# Autodesk Inventor assembly: XT-40
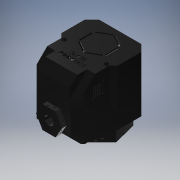
[picture p0: Inventor's stored thumbnail of the model, 180x180]
Saved by Autodesk Inventor 2017 SP1 (Build 210196100, 196)
## iProperties
Created: 2019-09-19
Part Number: XT-40
Document SubType Name: Assembly
Designer: Dell
Author: Dell
## Documents named in this file (17)
- C:\Users\Zach\Documents\GitHub\tr2\Actuator 2.0\XT-LG.iam
- C:\Users\Zach\Documents\GitHub\tr2\Actuator 2.0\AC01.ipt
- C:\Users\Zach\Documents\GitHub\tr2\Actuator 2.0\AC02.ipt
- C:\Users\Zach\Documents\GitHub\tr2\Actuator 2.0\AC05.ipt
- C:\Users\Zach\Documents\GitHub\tr2\Actuator 2.0\Slewing.iam
- C:\Users\Zach\Documents\GitHub\tr2\Actuator 2.0\Slip Ring.ipt
- C:\Users\Zach\Documents\GitHub\tr2\Actuator 2.0\8mm Mounting Hub.ipt
- C:\Users\Zach\Documents\GitHub\tr2\Actuator 2.0\AEAT-6012.ipt
- C:\Users\Zach\Documents\GitHub\tr2\Actuator 2.0\Series Elastic Gearbox 1.2\Series Elastic Gearbox 1.2.iam
- C:\Users\Zach\Documents\GitHub\tr2\Actuator 2.0\TS-40GZ7090.ipt
- C:\Users\Zach\Documents\GitHub\tr2\Actuator 2.0\Actuator 2.0\Design Accelerator\Spur Gears3.iam
- C:\Users\Zach\Documents\GitHub\tr2\Actuator 2.0\Actuator 2.0\Design Accelerator\Spur Gears4.iam
- C:\Users\Zach\Documents\GitHub\tr2\Actuator 2.0\Actuator 2.0\Design Accelerator\Spur Gears5.iam
- C:\Users\Zach\Documents\GitHub\tr2\Actuator 2.0\6201-2RS.ipt
- C:\Users\Zach\Documents\GitHub\tr2\Actuator 2.0\AC09.ipt
- C:\Users\Zach\Documents\GitHub\tr2\Actuator 2.0\AS 1110 - M6 x 35.ipt
- C:\Users\Zach\Documents\GitHub\tr2\Actuator 2.0\XT-LG-05.ipt
## Components (22 placed, 14 different names)
1. AC01:1 — Mate:3, Mate:4, Mate:5, Mate:9, Mate:139, Mate:140, Mate:141, Mate:142, Mate:145, Mate:146
2. AC02:1 — Mate:9, Mate:112, Mate:136, Mate:137, Mate:138, Mate:139, Mate:140, Mate:141, Mate:142, Mate:145, Mate:146, Mate:150, Mate:151, Mate:152, Mate:153, Mate:154, Mate:155, Mate:168, Mate:169, Mate:170, Mate:171, Mate:172, Mate:181, Mate:182, Mate:183, Mate:184, Flush:2, Flush:3
3. AC05:1 — Mate:6, Mate:7, Mate:8, Mate:23, Mate:24, Mate:25, Mate:90, Mate:91, Mate:92
4. Slewing:1 [sub-assembly] — Mate:3, Mate:4, Mate:5, Mate:6, Mate:7, Mate:8
5. Slip Ring:2 — Mate:23, Mate:24, Mate:25
6. 8mm Mounting Hub:1 — Mate:117, Mate:119
7. AEAT-6012:1 — Mate:151, Mate:158, Mate:162, Mate:163, Mate:164
8. AEAT-6012:2 — Mate:149, Mate:150, Mate:165, Mate:166, Mate:167
9. Series Elastic Gearbox 1.2:1 [sub-assembly] — Mate:90, Mate:91, Mate:92, Mate:113, Mate:114, Mate:116, Mate:120, Mate:134, Mate:143, Mate:156
10. TS-40GZ7090:1 — Mate:112, Mate:115, Mate:117, Mate:136, Mate:137, Mate:138, Mate:178, Mate:179, Mate:180
11. Spur Gears:1 [sub-assembly] — Mate:113, Mate:114, Mate:115, Mate:116, Mate:119, Mate:120, Rotation:1, Mate:144, Flush:1
12. Spur Gears:2 [sub-assembly] — Mate:134, Mate:143, Mate:144, Mate:156, Mate:158, Mate:174, Mate:177
13. Spur Gears:3 [sub-assembly] — Rotation:1, Mate:149, Flush:1, Mate:175, Mate:176
14. 6201-2RS:1 — Mate:154, Mate:155
15. 6201-2RS:2 — Mate:152, Mate:153
16. AC09:1 — Mate:162, Mate:163, Mate:164, Mate:165, Mate:166, Mate:167, Mate:168, Mate:169, Mate:170, Mate:171, Mate:172
17. AS 1110 - Metric M6 x 35:1 — Mate:174, Mate:177
18. AS 1110 - Metric M6 x 35:2 — Mate:175, Mate:176
19. AS 1110 - Metric M6 x 35:3 — Mate:178, Mate:181
20. AS 1110 - Metric M6 x 35:4 — Mate:179, Mate:182
21. AS 1110 - Metric M6 x 35:5 — Mate:180, Mate:183
22. XT-LG-05:1 — Mate:184, Flush:2, Flush:3
## Relationships (68: Mate 64, Flush 3, RelateRotation 1)
- Mate:3: AC01:1 ↔ Slewing:1
- Mate:4: AC01:1 ↔ Slewing:1
- Mate:5: AC01:1 ↔ Slewing:1
- Mate:6: AC05:1 ↔ Slewing:1
- Mate:7: AC05:1 ↔ Slewing:1
- Mate:8: AC05:1 ↔ Slewing:1
- Mate:9: AC01:1 ↔ AC02:1
- Mate:23: AC05:1 ↔ Slip Ring:2
- Mate:24 (5 mm): AC05:1 ↔ Slip Ring:2
- Mate:25: AC05:1 ↔ Slip Ring:2
- Mate:90: AC05:1 ↔ Series Elastic Gearbox 1.2:1
- Mate:91: AC05:1 ↔ Series Elastic Gearbox 1.2:1
- Mate:92: AC05:1 ↔ Series Elastic Gearbox 1.2:1
- Mate:112: AC02:1 ↔ TS-40GZ7090:1
- Mate:113: Series Elastic Gearbox 1.2:1 ↔ Spur Gears:1
- Mate:114: Series Elastic Gearbox 1.2:1 ↔ Spur Gears:1
- Mate:115: TS-40GZ7090:1 ↔ Spur Gears:1
- Mate:116: Series Elastic Gearbox 1.2:1 ↔ Spur Gears:1
- Mate:117: 8mm Mounting Hub:1 ↔ TS-40GZ7090:1
- Mate:119: 8mm Mounting Hub:1 ↔ Spur Gears:1
- Mate:120: Series Elastic Gearbox 1.2:1 ↔ Spur Gears:1
- Rotation:1 [RelateRotation] (1.0714 ul): Spur Gears:1 ↔ Spur Gears:3
- Mate:134: Series Elastic Gearbox 1.2:1 ↔ Spur Gears:2
- Mate:136: AC02:1 ↔ TS-40GZ7090:1
- Mate:137: AC02:1 ↔ TS-40GZ7090:1
- Mate:138: AC02:1 ↔ TS-40GZ7090:1
- Mate:139: AC01:1 ↔ AC02:1
- Mate:140: AC01:1 ↔ AC02:1
- Mate:141: AC01:1 ↔ AC02:1
- Mate:142: AC01:1 ↔ AC02:1
- Mate:143: Series Elastic Gearbox 1.2:1 ↔ Spur Gears:2
- Mate:144 (1 mm): Spur Gears:1 ↔ Spur Gears:2
- Mate:145: AC01:1 ↔ AC02:1
- Mate:146: AC01:1 ↔ AC02:1
- Mate:149: AEAT-6012:2 ↔ Spur Gears:3
- Flush:1: Spur Gears:1 ↔ Spur Gears:3
- Mate:150: AC02:1 ↔ AEAT-6012:2
- Mate:151: AC02:1 ↔ AEAT-6012:1
- Mate:152: AC02:1 ↔ 6201-2RS:2
- Mate:153: AC02:1 ↔ 6201-2RS:2
- Mate:154: AC02:1 ↔ 6201-2RS:1
- Mate:155: AC02:1 ↔ 6201-2RS:1
- Mate:156: Series Elastic Gearbox 1.2:1 ↔ Spur Gears:2
- Mate:158: AEAT-6012:1 ↔ Spur Gears:2
- Mate:162: AEAT-6012:1 ↔ AC09:1
- Mate:163: AEAT-6012:1 ↔ AC09:1
- Mate:164: AEAT-6012:1 ↔ AC09:1
- Mate:165: AEAT-6012:2 ↔ AC09:1
- Mate:166: AEAT-6012:2 ↔ AC09:1
- Mate:167: AEAT-6012:2 ↔ AC09:1
- Mate:168: AC02:1 ↔ AC09:1
- Mate:169: AC02:1 ↔ AC09:1
- Mate:170: AC02:1 ↔ AC09:1
- Mate:171: AC02:1 ↔ AC09:1
- Mate:172: AC02:1 ↔ AC09:1
- Mate:174: Spur Gears:2 ↔ AS 1110 - Metric M6 x 35:1
- Mate:175: Spur Gears:3 ↔ AS 1110 - Metric M6 x 35:2
- Mate:176: Spur Gears:3 ↔ AS 1110 - Metric M6 x 35:2
- Mate:177: Spur Gears:2 ↔ AS 1110 - Metric M6 x 35:1
- Mate:178: TS-40GZ7090:1 ↔ AS 1110 - Metric M6 x 35:3
- Mate:179: TS-40GZ7090:1 ↔ AS 1110 - Metric M6 x 35:4
- Mate:180: TS-40GZ7090:1 ↔ AS 1110 - Metric M6 x 35:5
- Mate:181: AC02:1 ↔ AS 1110 - Metric M6 x 35:3
- Mate:182: AC02:1 ↔ AS 1110 - Metric M6 x 35:4
- Mate:183: AC02:1 ↔ AS 1110 - Metric M6 x 35:5
- Mate:184: AC02:1 ↔ XT-LG-05:1
- Flush:2: AC02:1 ↔ XT-LG-05:1
- Flush:3: AC02:1 ↔ XT-LG-05:1
